# Autodesk Inventor assembly: MainAssembly
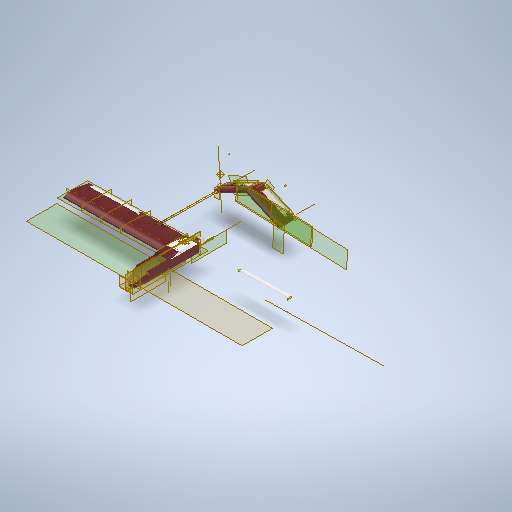
[picture p0: Inventor's stored thumbnail of the model, 512x512]
Saved by Autodesk Inventor 2026 (Build 300175050, 175E)
## iProperties
Created: 2025-08-01
Part Number: MainAssembly
Document SubType Name: Assembly
Designer: Cupri
Author: Cupri
## Documents named in this file (24)
- C:\Users\Cupri\OneDrive - University of South Carolina\UAV\SWIFT-UAV\System_development\Pelican\structural_model\v0.2.4\MainAssembly\MainAssembly.iam
- C:\Users\Cupri\OneDrive - University of South Carolina\UAV\SWIFT-UAV\System_development\Pelican\structural_model\v0.2.4\Parts\WingParts\WingBox.ipt
- C:\Users\Cupri\OneDrive - University of South Carolina\UAV\SWIFT-UAV\System_development\Pelican\structural_model\v0.2.4\Parts\WingParts\WingLeft_v0.1.ipt
- C:\Users\Cupri\OneDrive - University of South Carolina\UAV\SWIFT-UAV\System_development\Pelican\structural_model\v0.2.4\Parts\Extrusion\20x20x1295ExtrudedAluminum.ipt
- C:\Users\Cupri\OneDrive - University of South Carolina\UAV\SWIFT-UAV\System_development\Pelican\structural_model\v0.2.4\Parts\Extrusion\20x20x800ExtrudedAluminum.ipt
- C:\Users\Cupri\OneDrive - University of South Carolina\UAV\SWIFT-UAV\System_development\Pelican\structural_model\v0.2.4\Parts\MotorHousing.ipt
- C:\Users\Cupri\OneDrive - University of South Carolina\UAV\SWIFT-UAV\System_development\Pelican\structural_model\v0.2.4\Parts\Motor.ipt
- C:\Users\Cupri\OneDrive - University of South Carolina\UAV\SWIFT-UAV\System_development\Pelican\structural_model\v0.2.4\Parts\Fueselage.ipt
- C:\Users\Cupri\OneDrive - University of South Carolina\UAV\SWIFT-UAV\System_development\Pelican\structural_model\v0.2.4\Parts\FrontCover.ipt
- C:\Users\Cupri\OneDrive - University of South Carolina\UAV\SWIFT-UAV\System_development\Pelican\structural_model\v0.2.4\Parts\AlerionLeft.ipt
- C:\Users\Cupri\OneDrive - University of South Carolina\UAV\SWIFT-UAV\System_development\Pelican\structural_model\v0.2.4\Parts\Extrusion\20x20x1295ExtrudedAluminum_MIR.ipt
- C:\Users\Cupri\OneDrive - University of South Carolina\UAV\SWIFT-UAV\System_development\Pelican\structural_model\v0.2.4\Parts\WingParts\WingLeft_v0.1_MIR1.ipt
- C:\Users\Cupri\OneDrive - University of South Carolina\UAV\SWIFT-UAV\System_development\Pelican\structural_model\v0.2.4\Parts\Extrusion\20x20x800ExtrudedAluminum_MIR2.ipt
- C:\Users\Cupri\OneDrive - University of South Carolina\UAV\SWIFT-UAV\System_development\Pelican\structural_model\v0.2.4\Parts\Vtail.ipt
- C:\Users\Cupri\OneDrive - University of South Carolina\UAV\SWIFT-UAV\System_development\Pelican\structural_model\v0.2.4\Parts\Vtail_MIR.ipt
- C:\Users\Cupri\OneDrive - University of South Carolina\UAV\SWIFT-UAV\System_development\Pelican\structural_model\v0.2.4\Parts\AlerionLeft_MIR1.ipt
- C:\Users\Cupri\OneDrive - University of South Carolina\UAV\SWIFT-UAV\System_development\Pelican\structural_model\v0.2.4\Parts\Extrusion\20x20x785ExtrudedAluminum.ipt
- C:\Users\Cupri\OneDrive - University of South Carolina\UAV\SWIFT-UAV\System_development\Pelican\structural_model\v0.2.4\Parts\Mount v2.ipt
- C:\Users\Cupri\OneDrive - University of South Carolina\UAV\SWIFT-UAV\System_development\Pelican\structural_model\v0.2.4\Parts\kst-ds215mg-servo-1.snapshot.4\KST_DS215MG\KST_DS215MG\KST_DS215MG.ipt
- C:\Users\Cupri\OneDrive - University of South Carolina\UAV\SWIFT-UAV\System_development\Pelican\structural_model\v0.2.4\Parts\servo cap.ipt
- C:\Users\Cupri\OneDrive - University of South Carolina\UAV\SWIFT-UAV\System_development\Pelican\structural_model\v0.2.4\Parts\servo cap_MIR.ipt
- C:\Users\Cupri\OneDrive - University of South Carolina\UAV\SWIFT-UAV\System_development\Pelican\structural_model\v0.2.4\Parts\Tail.ipt
- C:\Users\Cupri\OneDrive - University of South Carolina\UAV\SWIFT-UAV\System_development\Pelican\structural_model\v0.2.4\Parts\Wing servo cap.ipt
- C:\Users\Cupri\OneDrive - University of South Carolina\UAV\SWIFT-UAV\System_development\Pelican\structural_model\v0.2.4\Parts\Wing servo cap_MIR1.ipt
## Components (24 placed, 23 different names)
1. Fueselage:1 — Mate:1, Mate:2, Flush:1, Flush:7, Mate:7, Flush:11, Mate:10, Mate:11, Mate:23, Angle:4, Mate:27, Mate:28, Mate:30, Mate:31, Mate:32, Flush:20
2. WingBox:1 — Mate:1, Mate:2, Mate:3, Angle:1, Flush:7
3. FrontCover:1 — Flush:1
4. 20x20x1295ExtrudedAluminum:1 — Mate:4, Mate:9
5. WingLeft_v0.1:1 — Mate:5, Angle:2, Mate:7, Rotational:1, Mate:47, Mate:52, Flush:19
6. 20x20x800ExtrudedAluminum:1 — Mate:9, Flush:12, Mate:51, Mate:52
7. MotorHousing:1 — Flush:11, Mate:10, Mate:11, Mate:12, Mate:13, Flush:16
8. Motor:1 — Mate:12, Mate:13
9. 20x20x1295ExtrudedAluminum_MIR:1 — Mate:16, Mate:19
10. WingLeft_v0.1_MIR1:1 — Mate:18, Angle:3
11. 20x20x800ExtrudedAluminum_MIR2:1 — Mate:19, Mate:49
12. Vtail:1 — Mate:41, Mate:42, Flush:17
13. Vtail_MIR:1 — Mate:44, Mate:45, Flush:18
14. AlerionLeft:1 — Rotational:1, Mate:48
15. AlerionLeft_MIR1:1
16. 20x20x785ExtrudedAluminum:1 — Mate:29, Mate:30, Mate:31, Mate:32
17. Mount v2:1 — Mate:25, Angle:6, Mate:27, Mate:28, Mate:29
18. KST_DS215MG:1 — Mate:47, Mate:48
19. KST_DS215MG:2 — Mate:53
20. servo cap:1
21. servo cap_MIR:1
22. Tail:1 — Mate:34, Mate:38, Mate:39, Mate:41, Mate:42, Mate:43, Angle:8, Mate:44, Mate:45, Mate:46, Angle:9, Mate:50, Mate:53
23. Wing servo cap:1 — Flush:19
24. Wing servo cap_MIR1:1
## Relationships (58: Mate 41, Flush 9, Angle 7, RevoluteJoint 1)
- Mate:1: Fueselage:1 ↔ WingBox:1
- Mate:2: Fueselage:1 ↔ WingBox:1
- Flush:1: Fueselage:1 ↔ FrontCover:1
- Mate:3: WingBox:1
- Angle:1 (0 deg): WingBox:1
- Mate:4: 20x20x1295ExtrudedAluminum:1
- Mate:5: WingLeft_v0.1:1
- Angle:2 (0 deg): WingLeft_v0.1:1
- Flush:7: Fueselage:1 ↔ WingBox:1
- Mate:6
- Mate:7: Fueselage:1 ↔ WingLeft_v0.1:1
- Mate:9: 20x20x1295ExtrudedAluminum:1 ↔ 20x20x800ExtrudedAluminum:1
- Flush:11: Fueselage:1 ↔ MotorHousing:1
- Mate:10: Fueselage:1 ↔ MotorHousing:1
- Mate:11: Fueselage:1 ↔ MotorHousing:1
- Mate:12: MotorHousing:1 ↔ Motor:1
- Mate:13: MotorHousing:1 ↔ Motor:1
- Mate:15
- Mate:16: 20x20x1295ExtrudedAluminum_MIR:1
- Mate:17
- Mate:18: WingLeft_v0.1_MIR1:1
- Angle:3 (0 deg): WingLeft_v0.1_MIR1:1
- Mate:19: 20x20x1295ExtrudedAluminum_MIR:1 ↔ 20x20x800ExtrudedAluminum_MIR2:1
- Flush:12 (-100 mm): 20x20x800ExtrudedAluminum:1
- Mate:23: Fueselage:1
- Rotational:1 [RevoluteJoint]: WingLeft_v0.1:1 ↔ AlerionLeft:1
- Flush:16 (50 mm): MotorHousing:1
- Angle:4 (0 deg): Fueselage:1
- Mate:25: Mount v2:1
- Angle:6 (0 deg): Mount v2:1
- Mate:27 (0.25 mm): Fueselage:1 ↔ Mount v2:1
- Mate:28 (23 mm): Fueselage:1 ↔ Mount v2:1
- Mate:29 (0.5 mm): 20x20x785ExtrudedAluminum:1 ↔ Mount v2:1
- Mate:30: Fueselage:1 ↔ 20x20x785ExtrudedAluminum:1
- Mate:31: Fueselage:1 ↔ 20x20x785ExtrudedAluminum:1
- Mate:32: Fueselage:1 ↔ 20x20x785ExtrudedAluminum:1
- Mate:34: Tail:1
- Mate:38: Tail:1
- Mate:39: Tail:1
- Mate:41: Vtail:1 ↔ Tail:1
- Mate:42: Vtail:1 ↔ Tail:1
- Mate:43: Tail:1
- Angle:8 (0 deg): Tail:1
- Flush:17: Vtail:1
- Mate:44: Vtail_MIR:1 ↔ Tail:1
- Mate:45: Vtail_MIR:1 ↔ Tail:1
- Mate:46: Tail:1
- Angle:9 (0 deg): Tail:1
- Flush:18: Vtail_MIR:1
- Mate:47: WingLeft_v0.1:1 ↔ KST_DS215MG:1
- Mate:48: AlerionLeft:1 ↔ KST_DS215MG:1
- Mate:49: 20x20x800ExtrudedAluminum_MIR2:1
- Mate:50: Tail:1
- Mate:51: 20x20x800ExtrudedAluminum:1
- Mate:52: WingLeft_v0.1:1 ↔ 20x20x800ExtrudedAluminum:1
- Mate:53 (0.25 mm): KST_DS215MG:2 ↔ Tail:1
- Flush:19: WingLeft_v0.1:1 ↔ Wing servo cap:1
- Flush:20: Fueselage:1
